# Autodesk Inventor assembly: Tank Tread Assembely
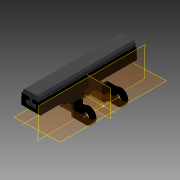
[picture p0: Inventor's stored thumbnail of the model, 180x180]
Saved by Autodesk Inventor 2015 (Build 190159000, 159)
## iProperties
Created: 2015-10-28
Part Number: Tank Tread Assembely
Document SubType Name: Assembly
Designer: Mason
Author: Mason
## Documents named in this file (3)
- C:\Users\User\Documents\Inventor\Content Center Files\FTC\Tank Tread Assembely.iam
- C:\Users\User\Documents\Inventor\Content Center Files\FTC\ASM parts DO NOT TOUCH\MAX Tank Tread Kit\tetrix_736468_tt_insert_2012.ipt
- C:\Users\User\Documents\Inventor\Content Center Files\FTC\ASM parts DO NOT TOUCH\MAX Tank Tread Kit\tetrix_736468_tt_link_2012.ipt
## Components (2 placed, 2 different names)
1. tetrix_736468_tt_link_2012:1 — Mate:1, Flush:1, Flush:2, Mate:2, Mate:3, Mate:4, Angle:1
2. tetrix_736468_tt_insert_2012:1 — Mate:1, Flush:1, Flush:2
## Relationships (7: Mate 4, Flush 2, Angle 1)
- Mate:1: tetrix_736468_tt_link_2012:1 ↔ tetrix_736468_tt_insert_2012:1
- Flush:1: tetrix_736468_tt_link_2012:1 ↔ tetrix_736468_tt_insert_2012:1
- Flush:2 (0.508 mm): tetrix_736468_tt_link_2012:1 ↔ tetrix_736468_tt_insert_2012:1
- Mate:2: tetrix_736468_tt_link_2012:1
- Mate:3: tetrix_736468_tt_link_2012:1
- Mate:4: tetrix_736468_tt_link_2012:1
- Angle:1 (90 deg): tetrix_736468_tt_link_2012:1
